# Autodesk Inventor assembly: SWEERVE V2
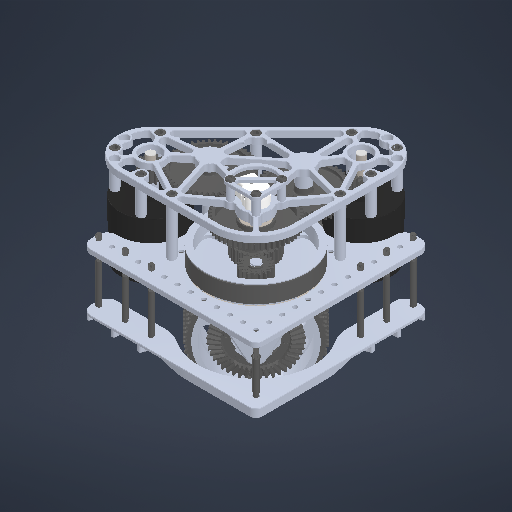
[picture p0: Inventor's stored thumbnail of the model, 512x512]
Saved by Autodesk Inventor 2026 (Build 300175000, 175)
## iProperties
Created: 2024-06-25
Part Number: SWEERVE V2
Document SubType Name: Assembly
Designer: gustavo.vieira
Mass: 6677.67 g
Surface Area: 4503.38 cm^2
Volume: 850.659 cm^3
Density: 7.85 g/cm^3
Author: gustavo.vieira
## Documents named in this file (24)
- C:\Users\DELL\OneDrive - SFIEMT\Área de Trabalho\FRC\FRC 2026\SWEERVE\SWEERVE V2.iam
- C:\Users\DELL\OneDrive - SFIEMT\Área de Trabalho\FRC\FRC 2026\SWEERVE\Screw, 10-32 X .25, Button, 91255A261_91255A261.ipt
- C:\Users\DELL\OneDrive - SFIEMT\Área de Trabalho\FRC\FRC 2026\SWEERVE\Screw, 10-32 X 1.5, 91251A351_91251A351.ipt
- C:\Users\DELL\OneDrive - SFIEMT\Área de Trabalho\FRC\FRC 2026\SWEERVE\Screw, 10-32 X 2.25, 91251A354_91251A354.ipt
- C:\Users\DELL\OneDrive - SFIEMT\Área de Trabalho\FRC\FRC 2026\SWEERVE\Screw, 8-32 X .875, Button, 91255A166_91255A166.ipt
- C:\Users\DELL\OneDrive - SFIEMT\Área de Trabalho\FRC\FRC 2026\SWEERVE\Bearing, 688.ipt
- C:\Users\DELL\OneDrive - SFIEMT\Área de Trabalho\FRC\FRC 2026\SWEERVE\Bearing, R188ZZ.ipt
- C:\Users\DELL\OneDrive - SFIEMT\Área de Trabalho\FRC\FRC 2026\SWEERVE\Gear, 50T, 20DP, .375Hex.ipt
- C:\Users\DELL\OneDrive - SFIEMT\Área de Trabalho\FRC\FRC 2026\SWEERVE\MK4i Steering Shaft Tall.ipt
- C:\Users\DELL\OneDrive - SFIEMT\Área de Trabalho\FRC\FRC 2026\SWEERVE\MK4i Steering Shaft Spacer.ipt
- C:\Users\DELL\OneDrive - SFIEMT\Área de Trabalho\FRC\FRC 2026\SWEERVE\MK4i Shaft, Drive Idler.ipt
- C:\Users\DELL\OneDrive - SFIEMT\Área de Trabalho\FRC\FRC 2026\SWEERVE\Screw, 3-48 X .1875, Pan Phillips, 90272A091_90272A091.ipt
- C:\Users\DELL\OneDrive - SFIEMT\Área de Trabalho\FRC\FRC 2026\SWEERVE\CANcoder Assembly.iam
- C:\Users\DELL\OneDrive - SFIEMT\Área de Trabalho\FRC\FRC 2026\SWEERVE\Motor, NEO.ipt
- C:\Users\DELL\OneDrive - SFIEMT\Área de Trabalho\FRC\FRC 2026\SWEERVE\Shim, 8mm ID X 14mm OD X .5mm Thick, 98055A115_98055A115.ipt
- C:\Users\DELL\OneDrive - SFIEMT\Área de Trabalho\FRC\FRC 2026\SWEERVE\Gear, 20DP, 14T, 8mm REV1.ipt
- C:\Users\DELL\OneDrive - SFIEMT\Área de Trabalho\FRC\FRC 2026\SWEERVE\Retaining Ring, 8mm, 98430A132_98430A132.ipt
- C:\Users\DELL\OneDrive - SFIEMT\Área de Trabalho\FRC\FRC 2026\SWEERVE\Spacer, 8mmID X .437 OD X 0.437 L.ipt
- C:\Users\DELL\OneDrive - SFIEMT\Área de Trabalho\FRC\FRC 2026\SWEERVE\Machine Key, 2 X 2 X 12mm.ipt
- C:\Users\DELL\OneDrive - SFIEMT\Área de Trabalho\FRC\FRC 2026\SWEERVE\Belt, 320-5M-15.ipt
- C:\Users\DELL\OneDrive - SFIEMT\Área de Trabalho\FRC\FRC 2026\SWEERVE\MK4 Turret Assembly_Billet Wheel.iam
- C:\Users\DELL\OneDrive - SFIEMT\Área de Trabalho\FRC\FRC 2026\SWEERVE\MK4i Master Part V2_NEO Config.ipt
- C:\Users\DELL\OneDrive - SFIEMT\Área de Trabalho\FRC\FRC 2026\SWEERVE\Screw, 10-32 X 2.5, 91251A355_91251A355.ipt
- C:\Users\DELL\OneDrive - SFIEMT\Área de Trabalho\FRC\FRC 2026\SWEERVE\MK4i Master Part V3_NEO Config.ipt
## Components (50 placed, 23 different names)
1. Screw, 10-32 X .25, Button, 91255A261_91255A261:1
2. Screw, 10-32 X .25, Button, 91255A261_91255A261:2
3. Screw, 10-32 X .25, Button, 91255A261_91255A261:3
4. Screw, 10-32 X .25, Button, 91255A261_91255A261:4
5. Screw, 10-32 X .25, Button, 91255A261_91255A261:5
6. Screw, 10-32 X 1.5, 91251A351_91251A351:1
7. Screw, 10-32 X 2.25, 91251A354_91251A354:1
8. Screw, 10-32 X 2.25, 91251A354_91251A354:2
9. Screw, 10-32 X 2.25, 91251A354_91251A354:3
10. Screw, 10-32 X 2.25, 91251A354_91251A354:4 — Coincidente:7, Coincidente:17
11. Screw, 8-32 X .875, Button, 91255A166_91255A166:1
12. Screw, 8-32 X .875, Button, 91255A166_91255A166:2
13. Screw, 8-32 X .875, Button, 91255A166_91255A166:3
14. Bearing, 688:2
15. Bearing, R188ZZ:1
16. Bearing, 688:3
17. Bearing, 688:4
18. Gear, 50T, 20DP, .375Hex:1
19. Gear, 50T, 20DP, .375Hex:2
20. MK4i Steering Shaft Tall:1
21. MK4i Steering Shaft Spacer:1
22. MK4i Shaft, Drive Idler:1
23. Screw, 3-48 X .1875, Pan Phillips, 90272A091_90272A091:1
24. CANcoder Assembly:1 [sub-assembly]
25. Screw, 3-48 X .1875, Pan Phillips, 90272A091_90272A091:2
26. Motor, NEO:1
27. Motor, NEO:2
28. Shim, 8mm ID X 14mm OD X .5mm Thick, 98055A115_98055A115:2
29. Gear, 20DP, 14T, 8mm REV1:1
30. Retaining Ring, 8mm, 98430A132_98430A132:1
31. Gear, 20DP, 14T, 8mm REV1:2
32. Spacer, 8mmID X .437 OD X 0.437 L:1
33. Retaining Ring, 8mm, 98430A132_98430A132:2
34. Machine Key, 2 X 2 X 12mm:1
35. Machine Key, 2 X 2 X 12mm:2
36. Belt, 320-5M-15:1
37. Screw, 10-32 X 1.5, 91251A351_91251A351:2
38. Screw, 10-32 X 1.5, 91251A351_91251A351:3
39. Screw, 10-32 X 1.5, 91251A351_91251A351:4
40. Screw, 10-32 X 1.5, 91251A351_91251A351:5
41. Screw, 10-32 X 1.5, 91251A351_91251A351:6
42. MK4 Turret Assembly_Billet Wheel:1 [sub-assembly]
43. MK4i Master Part V2_NEO Config:1 — Coincidente:1, Coincidente:2, Coincidente:3
44. Screw, 10-32 X 2.5, 91251A355_91251A355:1 — Coincidente:9, Coincidente:12
45. Screw, 10-32 X 2.5, 91251A355_91251A355:2 — Coincidente:8, Coincidente:13
46. Screw, 10-32 X 2.5, 91251A355_91251A355:3 — Coincidente:4, Coincidente:14
47. Screw, 10-32 X 2.5, 91251A355_91251A355:4 — Coincidente:5, Coincidente:15
48. Screw, 10-32 X 2.5, 91251A355_91251A355:5 — Coincidente:6, Coincidente:16
49. Screw, 10-32 X 2.5, 91251A355_91251A355:6 — Coincidente:10, Coincidente:11
50. MK4i Master Part V3_NEO Config:1 — Coincidente:1, Coincidente:2, Coincidente:3, Coincidente:4, Coincidente:5, Coincidente:6, Coincidente:7, Coincidente:8, Coincidente:9, Coincidente:10, Coincidente:11, Coincidente:12, Coincidente:13, Coincidente:14, Coincidente:15, Coincidente:16, Coincidente:17
## Relationships (17: Mate 17)
- Coincidente:1 [Mate]: MK4i Master Part V2_NEO Config:1 ↔ MK4i Master Part V3_NEO Config:1
- Coincidente:2 [Mate]: MK4i Master Part V2_NEO Config:1 ↔ MK4i Master Part V3_NEO Config:1
- Coincidente:3 [Mate] (50.8 mm): MK4i Master Part V2_NEO Config:1 ↔ MK4i Master Part V3_NEO Config:1
- Coincidente:4 [Mate]: Screw, 10-32 X 2.5, 91251A355_91251A355:3 ↔ MK4i Master Part V3_NEO Config:1
- Coincidente:5 [Mate]: Screw, 10-32 X 2.5, 91251A355_91251A355:4 ↔ MK4i Master Part V3_NEO Config:1
- Coincidente:6 [Mate]: Screw, 10-32 X 2.5, 91251A355_91251A355:5 ↔ MK4i Master Part V3_NEO Config:1
- Coincidente:7 [Mate]: Screw, 10-32 X 2.25, 91251A354_91251A354:4 ↔ MK4i Master Part V3_NEO Config:1
- Coincidente:8 [Mate]: Screw, 10-32 X 2.5, 91251A355_91251A355:2 ↔ MK4i Master Part V3_NEO Config:1
- Coincidente:9 [Mate]: Screw, 10-32 X 2.5, 91251A355_91251A355:1 ↔ MK4i Master Part V3_NEO Config:1
- Coincidente:10 [Mate]: Screw, 10-32 X 2.5, 91251A355_91251A355:6 ↔ MK4i Master Part V3_NEO Config:1
- Coincidente:11 [Mate]: Screw, 10-32 X 2.5, 91251A355_91251A355:6 ↔ MK4i Master Part V3_NEO Config:1
- Coincidente:12 [Mate]: Screw, 10-32 X 2.5, 91251A355_91251A355:1 ↔ MK4i Master Part V3_NEO Config:1
- Coincidente:13 [Mate]: Screw, 10-32 X 2.5, 91251A355_91251A355:2 ↔ MK4i Master Part V3_NEO Config:1
- Coincidente:14 [Mate]: Screw, 10-32 X 2.5, 91251A355_91251A355:3 ↔ MK4i Master Part V3_NEO Config:1
- Coincidente:15 [Mate]: Screw, 10-32 X 2.5, 91251A355_91251A355:4 ↔ MK4i Master Part V3_NEO Config:1
- Coincidente:16 [Mate]: Screw, 10-32 X 2.5, 91251A355_91251A355:5 ↔ MK4i Master Part V3_NEO Config:1
- Coincidente:17 [Mate]: Screw, 10-32 X 2.25, 91251A354_91251A354:4 ↔ MK4i Master Part V3_NEO Config:1
